# Autodesk Inventor assembly: Wheel Coupler Assembly
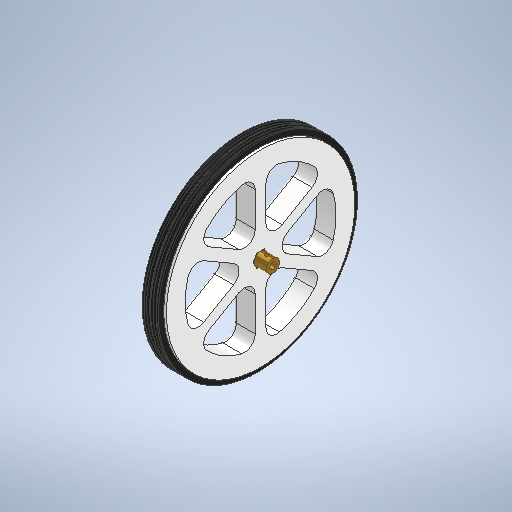
[picture p0: Inventor's stored thumbnail of the model, 512x512]
Saved by Autodesk Inventor 2025.2 (Build 292293000, 293)
## iProperties
Created: 2025-02-25
Part Number: Wheel Coupler Assembly
Document SubType Name: Assembly
Designer: Matt Tidd
Mass: 298.9 g
Surface Area: 906.457 cm^2
Volume: 298.9 cm^3
Density: 1 g/cm^3
Author: Matt Tidd
## Documents named in this file (4)
- C:\Users\mtidd2\Desktop\H2A\CAD\Motors_and_Wheels\Wheel Assembly\Wheel Coupler Assembly.iam
- C:\Users\mtidd2\Desktop\H2A\CAD\Motors_and_Wheels\Wheel Assembly\520 DC Gear Motor Wheel Coupler.ipt
- C:\Users\mtidd2\Desktop\H2A\CAD\Motors_and_Wheels\Wheel Assembly\PLA Wheel Frame.ipt
- C:\Users\mtidd2\Desktop\H2A\CAD\Motors_and_Wheels\Wheel Assembly\TPU Tire.ipt
## Components (3 placed, 3 different names)
1. PLA Wheel Frame:1 — Flush:3, Mate:1, Mate:2, Mate:3
2. TPU Tire:1 — Mate:2, Mate:3
3. 520 DC Gear Motor Wheel Coupler:1 — Mate:1
## Relationships (6: Flush 3, Mate 3)
- [Flush]: PLA Wheel Frame:1
- [Flush]: PLA Wheel Frame:1
- Flush:3: PLA Wheel Frame:1
- Mate:1: PLA Wheel Frame:1 ↔ 520 DC Gear Motor Wheel Coupler:1
- Mate:2: PLA Wheel Frame:1 ↔ TPU Tire:1
- Mate:3: PLA Wheel Frame:1 ↔ TPU Tire:1
